# Autodesk Inventor assembly: base_ass_1
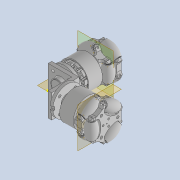
[picture p0: Inventor's stored thumbnail of the model, 180x180]
Saved by Autodesk Inventor 2020 (Build 240168000, 168)
## iProperties
Created: 2022-01-11
Part Number: base_ass_1
Document SubType Name: Assembly
Designer: Shuang Peng
Author: Shuang Peng
## Documents named in this file (6)
- D:\projects-3\soft module robot\hardware\diff module 3\base_ass_1.iam
- D:\projects-3\soft module robot\hardware\diff module 3\motor_1613_2.iam
- D:\projects-3\soft module robot\hardware\diff module 3\base_1.ipt
- D:\projects-3\soft module robot\hardware\diff module 3\wheel_ass_2.iam
- D:\projects-3\soft module robot\hardware\diff module 3\ma_holder_1.ipt
- D:\projects-3\soft module robot\hardware\diff module 3\encoder_ma_6_2.5.ipt
## Components (9 placed, 5 different names)
1. motor_1613_2:1 [sub-assembly] — Angle:1, Flush:1, Flush:2, Flush:3, Flush:4, Insert:1, Insert:2, Flush:7, Insert:5, Insert:8
2. motor_1613_2:2 [sub-assembly] — Angle:1, Flush:1, Flush:2, Flush:3, Insert:3, Insert:4, Insert:9
3. base_1:1 — Flush:5, Flush:6, Insert:8
4. wheel_ass_2:1 [sub-assembly] — Insert:3, Insert:4
5. wheel_ass_2:2 [sub-assembly] — Insert:1, Insert:2
6. ma_holder_1:1 — Flush:7, Insert:5, Insert:6
7. encoder_ma_6_2.5:1 — Insert:6
8. ma_holder_1:2 — Insert:9
9. encoder_ma_6_2.5:2
## Relationships (17: Insert 9, Flush 7, Angle 1)
- Angle:1 (-90 deg): motor_1613_2:1 ↔ motor_1613_2:2
- Flush:1: motor_1613_2:1 ↔ motor_1613_2:2
- Flush:2 (-13.5 mm): motor_1613_2:1 ↔ motor_1613_2:2
- Flush:3 (-13.5 mm): motor_1613_2:1 ↔ motor_1613_2:2
- Flush:4 (-5.5 mm): motor_1613_2:1
- Flush:5: base_1:1
- Flush:6: base_1:1
- Insert:1: motor_1613_2:1 ↔ wheel_ass_2:2
- Insert:2: motor_1613_2:1 ↔ wheel_ass_2:2
- Insert:3: motor_1613_2:2 ↔ wheel_ass_2:1
- Insert:4: motor_1613_2:2 ↔ wheel_ass_2:1
- Flush:7: motor_1613_2:1 ↔ ma_holder_1:1
- Insert:5 (-0.5 mm): motor_1613_2:1 ↔ ma_holder_1:1
- Insert:6: ma_holder_1:1 ↔ encoder_ma_6_2.5:1
- [Insert]: ma_holder_1:2 ↔ encoder_ma_6_2.5:2
- Insert:8: motor_1613_2:1 ↔ base_1:1
- Insert:9 (-0.5 mm): motor_1613_2:2 ↔ ma_holder_1:2
## Named parameters: d18_d17 = 0 mm
